# Autodesk Inventor assembly: IdealGasAssembly
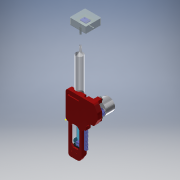
[picture p0: Inventor's stored thumbnail of the model, 180x180]
Saved by Autodesk Inventor 2018 (Build 220112000, 112)
## iProperties
Created: 2020-02-29
Part Number: IdealGasAssembly
Document SubType Name: Assembly
Designer: Ivan
Author: Ivan
## Documents named in this file (13)
- C:\Users\Ivan\Documents\GitHub\IdealGas\3D Model\IdealGasAssembly.iam
- C:\Users\Ivan\Documents\GitHub\IdealGas\3D Model\Base.ipt
- C:\Users\Ivan\Documents\GitHub\IdealGas\3D Model\MotorGear.ipt
- C:\Users\Ivan\Documents\GitHub\IdealGas\3D Model\Pinon.ipt
- C:\Users\Ivan\Documents\GitHub\IdealGas\3D Model\Rack.ipt
- C:\Users\Ivan\Documents\GitHub\IdealGas\3D Model\Geared Stepper.ipt
- C:\Users\Ivan\Documents\GitHub\IdealGas\3D Model\syringe_body.ipt
- C:\Users\Ivan\Documents\GitHub\IdealGas\3D Model\syringe_piston.ipt
- C:\Users\Ivan\Documents\GitHub\IdealGas\3D Model\syringe_plunger.ipt
- C:\Users\Ivan\Documents\Inventor\Content Center Files\R2018\en-US\ASME ANSI B18.3.5M(2)\ASME_ANSI B18.3.5M - M4x10(2).ipt
- C:\Users\Ivan\Documents\GitHub\IdealGas\3D Model\Limit_Switch.ipt
- C:\Users\Ivan\Documents\GitHub\IdealGas\3D Model\DAQcapsule.ipt
- C:\Users\Ivan\Documents\GitHub\IdealGas\3D Model\BMP180.ipt
## Components (13 placed, 12 different names)
1. Base:1 — Insert:3, Angle:1, Insert:4, Mate:4, Angle:2, Mate:5, Insert:5, Angle:3, Angle:4, Mate:7, Mate:8, Mate:9, Mate:10, Mate:11, Mate:14, Angle:5, Angle:6
2. syringe_body:1 — Insert:2, Insert:5, Angle:3, Mate:15
3. syringe_piston:1 — Insert:1
4. syringe_plunger:1 — Insert:1, Insert:2, Mate:6, Angle:4
5. Geared Stepper:1 — Mate:1, Mate:2, Mate:3, Insert:3, Angle:1
6. Rack:1 — Mate:4, Angle:2, Mate:5, Mate:6, Rotation/Translation:1
7. MotorGear:1 — Mate:1, Mate:2, Mate:3
8. Pinon:1 — Insert:4, Rotation/Translation:1
9. Broached Hexagon Socket Flat Countersunk Head Cap Screws - Metric M4x10:1 — Mate:7
10. Broached Hexagon Socket Flat Countersunk Head Cap Screws - Metric M4x10:2 — Mate:8
11. Limit_Switch:1 — Mate:9, Mate:10, Mate:11
12. DAQcapsule:1 — Mate:12, Mate:13, Mate:14, Angle:6, Mate:15
13. BMP180:1 — Mate:12, Mate:13, Angle:5
## Relationships (27: Mate 15, Angle 6, Insert 5, RelateRotateTranslate 1)
- Insert:1: syringe_piston:1 ↔ syringe_plunger:1
- Insert:2 (8 mm): syringe_body:1 ↔ syringe_plunger:1
- Mate:1: Geared Stepper:1 ↔ MotorGear:1
- Mate:2: Geared Stepper:1 ↔ MotorGear:1
- Mate:3: Geared Stepper:1 ↔ MotorGear:1
- Insert:3: Base:1 ↔ Geared Stepper:1
- Angle:1 (0 deg): Base:1 ↔ Geared Stepper:1
- Insert:4: Base:1 ↔ Pinon:1
- Mate:4: Base:1 ↔ Rack:1
- Angle:2 (0 deg): Base:1 ↔ Rack:1
- Mate:5: Base:1 ↔ Rack:1
- Insert:5 (-10 mm): Base:1 ↔ syringe_body:1
- Angle:3 (0 deg): Base:1 ↔ syringe_body:1
- Mate:6: syringe_plunger:1 ↔ Rack:1
- Rotation/Translation:1 [RelateRotateTranslate] (200 mm): Rack:1 ↔ Pinon:1
- Angle:4 (0 deg): Base:1 ↔ syringe_plunger:1
- Mate:7: Base:1 ↔ Broached Hexagon Socket Flat Countersunk Head Cap Screws - Metric M4x10:1
- Mate:8: Base:1 ↔ Broached Hexagon Socket Flat Countersunk Head Cap Screws - Metric M4x10:2
- Mate:9: Base:1 ↔ Limit_Switch:1
- Mate:10: Base:1 ↔ Limit_Switch:1
- Mate:11: Base:1 ↔ Limit_Switch:1
- Mate:12: DAQcapsule:1 ↔ BMP180:1
- Mate:13: DAQcapsule:1 ↔ BMP180:1
- Mate:14 (120 mm): Base:1 ↔ DAQcapsule:1
- Angle:5 (0 deg): Base:1 ↔ BMP180:1
- Angle:6 (0 deg): Base:1 ↔ DAQcapsule:1
- Mate:15: syringe_body:1 ↔ DAQcapsule:1
